# Autodesk Inventor assembly: shaft and nut
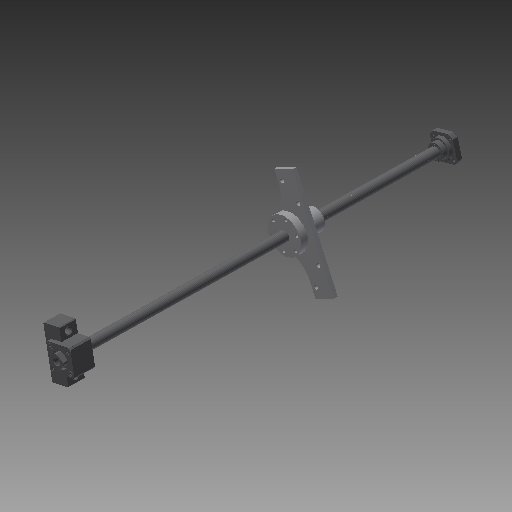
[picture p0: Inventor's stored thumbnail of the model, 512x512]
Saved by Autodesk Inventor 2018 (Build 220112000, 112)
## iProperties
Created: 2017-06-20
Part Number: shaft and nut
Document SubType Name: Assembly
Designer: M228544
Author: M228544
## Documents named in this file (7)
- C:\Users\P301319\Documents\GitHub\CNC-Lathe-CAD\2018\short shaft x axis\shaft and nut.iam
- C:\Users\P301319\Documents\GitHub\CNC-Lathe-CAD\2018\short shaft x axis\nut.ipt
- C:\Users\P301319\Documents\GitHub\CNC-Lathe-CAD\2018\short shaft x axis\shaft.ipt
- C:\Users\P301319\Documents\GitHub\CNC-Lathe-CAD\2018\short shaft x axis\FF 10Part1.ipt
- C:\Users\P301319\Documents\GitHub\CNC-Lathe-CAD\2018\short shaft x axis\EK 10.ipt
- C:\Users\P301319\Documents\GitHub\CNC-Lathe-CAD\2018\short shaft x axis\FF 10 Part2.ipt
- C:\Users\P301319\Documents\GitHub\CNC-Lathe-CAD\2018\short shaft x axis\x axis nut support.ipt
## Components (6 placed, 6 different names)
1. nut:1 — Mate:12, Mate:13, Mate:14
2. shaft:1 — Mate:2, Mate:3, Mate:4, Mate:6, Mate:7, Mate:11, Mate:12
3. FF 10Part1:1 — Mate:8, Mate:9
4. EK 10:1 — Mate:2, Mate:3, Mate:7
5. FF 10 Part2:1 — Mate:4, Mate:6, Mate:8, Mate:9
6. x axis nut support-01:1 — Mate:11, Mate:13, Mate:14
## Relationships (11: Mate 11)
- Mate:2: shaft:1 ↔ EK 10:1
- Mate:3: shaft:1 ↔ EK 10:1
- Mate:4: shaft:1 ↔ FF 10 Part2:1
- Mate:6: shaft:1 ↔ FF 10 Part2:1
- Mate:7: shaft:1 ↔ EK 10:1
- Mate:8: FF 10Part1:1 ↔ FF 10 Part2:1
- Mate:9: FF 10Part1:1 ↔ FF 10 Part2:1
- Mate:11: shaft:1 ↔ x axis nut support-01:1
- Mate:12: nut:1 ↔ shaft:1
- Mate:13: nut:1 ↔ x axis nut support-01:1
- Mate:14: nut:1 ↔ x axis nut support-01:1
